# Autodesk Inventor assembly: right_part_MIR
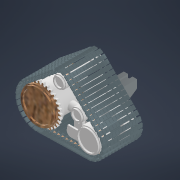
[picture p0: Inventor's stored thumbnail of the model, 180x180]
Saved by Autodesk Inventor 2022 (Build 260153000, 153)
## iProperties
Created: 2021-12-31
Part Number: right_part_MIR
Document SubType Name: Assembly
Designer: MatusBarany
Author: MatusBarany
## Documents named in this file (12)
- C:\Users\MatusBarany\Documents\Inventor\wall-e\matus\right_part_MIR.iam
- C:\Users\Public\Documents\Autodesk\Inventor 2022\Projects\wall-e\wheel connector_MIR.ipt
- C:\Users\Public\Documents\Autodesk\Inventor 2022\Projects\wall-e\under walle L3_MIR.ipt
- C:\Users\Public\Documents\Autodesk\Inventor 2022\Projects\wall-e\uchytka_spojky_medzi_velkym_strednym_MIR.ipt
- C:\Users\Public\Documents\Autodesk\Inventor 2022\Projects\wall-e\spojka_pol_velke_koleso_MIR.ipt
- C:\Users\Public\Documents\Autodesk\Inventor 2022\Projects\wall-e\spojka_pol_stredne_koleso_MIR.ipt
- C:\Users\Public\Documents\Autodesk\Inventor 2022\Projects\wall-e\velke_koleso_MIR.ipt
- C:\Users\Public\Documents\Autodesk\Inventor 2022\Projects\wall-e\stredne_koleso_MIR.ipt
- C:\Users\Public\Documents\Autodesk\Inventor 2022\Projects\wall-e\male_koliesko_MIR.ipt
- C:\Users\Public\Documents\Autodesk\Inventor 2022\Projects\wall-e\spojka_male_koleso_MIR.ipt
- C:\Users\Public\Documents\Autodesk\Inventor 2022\Projects\wall-e\chain right_MIR.ipt
- C:\Users\Public\Documents\Autodesk\Inventor 2022\Projects\wall-e\onePart_chain_MIR.ipt
## Components (68 placed, 11 different names)
1. wheel connector_MIR:1 — Mate:3, Mate:2, Mate:1, Mate:6, Mate:5, Mate:4, Rotational:1
2. under walle L3_MIR:1 — Mate:3, Mate:2, Mate:1
3. uchytka_spojky_medzi_velkym_strednym_MIR:1 — Mate:6, Mate:5, Mate:4, Mate:7, Cylindrical:1
4. spojka_pol_velke_koleso_MIR:1 — Mate:7, Flush:2, Flush:1, Mate:8, Cylindrical:1, Rigid:1, Rigid:2
5. spojka_pol_stredne_koleso_MIR:1 — Flush:2, Flush:1, Mate:8, Rigid:3, Rigid:4
6. velke_koleso_MIR:1 — Flush:3, Rigid:1
7. velke_koleso_MIR:2 — Rigid:2
8. stredne_koleso_MIR:1 — Rigid:3
9. stredne_koleso_MIR:2 — Rigid:4
10. male_koliesko_MIR:1 — Rigid:6
11. male_koliesko_MIR:2 — Rigid:9
12. male_koliesko_MIR:3 — Rigid:8
13. male_koliesko_MIR:4 — Rigid:7
14. spojka_male_koleso_MIR:1 — Rotational:1, Rigid:9, Rigid:8, Rigid:7, Rigid:6
15. chain right_MIR:1 — Mate:10, Mate:9, Flush:6, Flush:5, Flush:4
16. onePart_chain_MIR:1 — Mate:10, Mate:9, Flush:6
17. onePart_chain_MIR:2
18. onePart_chain_MIR:3
19. onePart_chain_MIR:4
20. onePart_chain_MIR:5
21. onePart_chain_MIR:6
22. onePart_chain_MIR:7
23. onePart_chain_MIR:8
24. onePart_chain_MIR:9
25. onePart_chain_MIR:10
26. onePart_chain_MIR:11
27. onePart_chain_MIR:12
28. onePart_chain_MIR:13
29. onePart_chain_MIR:14
30. onePart_chain_MIR:15
31. onePart_chain_MIR:16
32. onePart_chain_MIR:17
33. onePart_chain_MIR:18
34. onePart_chain_MIR:19
35. onePart_chain_MIR:20
36. onePart_chain_MIR:21
37. onePart_chain_MIR:22
38. onePart_chain_MIR:23
39. onePart_chain_MIR:24
40. onePart_chain_MIR:25
41. onePart_chain_MIR:26
42. onePart_chain_MIR:27
43. onePart_chain_MIR:28
44. onePart_chain_MIR:29
45. onePart_chain_MIR:30
46. onePart_chain_MIR:31
47. onePart_chain_MIR:32
48. onePart_chain_MIR:33
49. onePart_chain_MIR:34
50. onePart_chain_MIR:35
51. onePart_chain_MIR:36
52. onePart_chain_MIR:37
53. onePart_chain_MIR:38
54. onePart_chain_MIR:39
55. onePart_chain_MIR:40
56. onePart_chain_MIR:41
57. onePart_chain_MIR:42
58. onePart_chain_MIR:43
59. onePart_chain_MIR:44
60. onePart_chain_MIR:45
61. onePart_chain_MIR:46
62. onePart_chain_MIR:47
63. onePart_chain_MIR:48
64. onePart_chain_MIR:49
65. onePart_chain_MIR:50
66. onePart_chain_MIR:51
67. onePart_chain_MIR:52
68. onePart_chain_MIR:53
## Relationships (26: Mate 12, WeldJoint 8, Flush 4, CylindricalJoint 1, RevoluteJoint 1)
- Mate:3: wheel connector_MIR:1 ↔ under walle L3_MIR:1
- Mate:2: wheel connector_MIR:1 ↔ under walle L3_MIR:1
- Mate:1: wheel connector_MIR:1 ↔ under walle L3_MIR:1
- Mate:6: wheel connector_MIR:1 ↔ uchytka_spojky_medzi_velkym_strednym_MIR:1
- Mate:5: wheel connector_MIR:1 ↔ uchytka_spojky_medzi_velkym_strednym_MIR:1
- Mate:4: wheel connector_MIR:1 ↔ uchytka_spojky_medzi_velkym_strednym_MIR:1
- Mate:7: uchytka_spojky_medzi_velkym_strednym_MIR:1 ↔ spojka_pol_velke_koleso_MIR:1
- Flush:2: spojka_pol_velke_koleso_MIR:1 ↔ spojka_pol_stredne_koleso_MIR:1
- Flush:1: spojka_pol_velke_koleso_MIR:1 ↔ spojka_pol_stredne_koleso_MIR:1
- Mate:8: spojka_pol_velke_koleso_MIR:1 ↔ spojka_pol_stredne_koleso_MIR:1
- Flush:3 (-1.5 mm): velke_koleso_MIR:1
- Mate:10: chain right_MIR:1 ↔ onePart_chain_MIR:1
- Mate:9: chain right_MIR:1 ↔ onePart_chain_MIR:1
- Flush:6: chain right_MIR:1 ↔ onePart_chain_MIR:1
- Flush:5 [Mate]: chain right_MIR:1
- Flush:4 [Mate]: chain right_MIR:1
- Cylindrical:1: uchytka_spojky_medzi_velkym_strednym_MIR:1 ↔ spojka_pol_velke_koleso_MIR:1
- Rigid:1 [WeldJoint]: spojka_pol_velke_koleso_MIR:1 ↔ velke_koleso_MIR:1
- Rigid:2 [WeldJoint]: spojka_pol_velke_koleso_MIR:1 ↔ velke_koleso_MIR:2
- Rigid:3 [WeldJoint]: spojka_pol_stredne_koleso_MIR:1 ↔ stredne_koleso_MIR:1
- Rigid:4 [WeldJoint]: spojka_pol_stredne_koleso_MIR:1 ↔ stredne_koleso_MIR:2
- Rotational:1 [RevoluteJoint]: wheel connector_MIR:1 ↔ spojka_male_koleso_MIR:1
- Rigid:9 [WeldJoint]: male_koliesko_MIR:2 ↔ spojka_male_koleso_MIR:1
- Rigid:8 [WeldJoint]: male_koliesko_MIR:3 ↔ spojka_male_koleso_MIR:1
- Rigid:7 [WeldJoint]: male_koliesko_MIR:4 ↔ spojka_male_koleso_MIR:1
- Rigid:6 [WeldJoint]: male_koliesko_MIR:1 ↔ spojka_male_koleso_MIR:1
